# Autodesk Inventor assembly: Dome
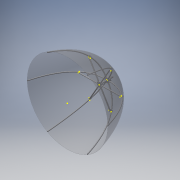
[picture p0: Inventor's stored thumbnail of the model, 180x180]
Saved by Autodesk Inventor 2018 (Build 220112000, 112)
## iProperties
Created: 2019-06-02
Part Number: Dome
Document SubType Name: Assembly
Designer: dell
Author: dell
## Documents named in this file (7)
- C:\Users\dell\Desktop\IITD stuff\DISA\Dome.iam
- C:\Users\dell\Desktop\IITD stuff\DISA\Holder.ipt
- C:\Users\dell\Desktop\IITD stuff\DISA\Rib.ipt
- C:\Users\dell\Desktop\IITD stuff\DISA\Covering.ipt
- C:\Users\dell\Desktop\IITD stuff\DISA\PropUp.ipt
- C:\Users\dell\Desktop\IITD stuff\DISA\Joiner.ipt
- C:\Users\dell\Desktop\IITD stuff\DISA\Screw.ipt
## Components (21 placed, 6 different names)
1. Holder:1 — Mate:1, Mate:2, Mate:3, Mate:4, Mate:5, Mate:6, Flush:1, Insert:1
2. Rib:1 — Mate:1, Angle:5
3. Rib:2 — Mate:2, Angle:6
4. Rib:3 — Mate:3, Angle:1
5. Rib:4 — Mate:4, Angle:2
6. Rib:5 — Mate:5, Angle:3
7. Rib:6 — Mate:6, Angle:4
8. Covering:1 — Angle:7
9. PropUp:1 — Angle:8, Insert:1, Insert:2
10. Joiner:1
11. Joiner:7
12. Joiner:8
13. Joiner:9
14. Joiner:10
15. Joiner:11
16. Screw:1 — Insert:2
17. Screw:2
18. Screw:3
19. Screw:4
20. Screw:5
21. Screw:6
## Component patterns: (6 elements, first: Joiner:1), (6 elements, first: Screw:1)
## Relationships (17: Angle 8, Mate 6, Insert 2, Flush 1)
- Mate:1: Holder:1 ↔ Rib:1
- Mate:2: Holder:1 ↔ Rib:2
- Mate:3: Holder:1 ↔ Rib:3
- Mate:4: Holder:1 ↔ Rib:4
- Mate:5: Holder:1 ↔ Rib:5
- Mate:6: Holder:1 ↔ Rib:6
- Flush:1 (-800 mm): Holder:1
- Angle:1 (0 deg): Rib:3
- Angle:2 (0 deg): Rib:4
- Angle:3 (0 deg): Rib:5
- Angle:4 (0 deg): Rib:6
- Angle:5 (0 deg): Rib:1
- Angle:6 (0 deg): Rib:2
- Angle:7 (0 deg): Covering:1
- Angle:8 (0 deg): PropUp:1
- Insert:1: Holder:1 ↔ PropUp:1
- Insert:2 (7.5 mm): PropUp:1 ↔ Screw:1
